# Autodesk Inventor assembly: 305-05
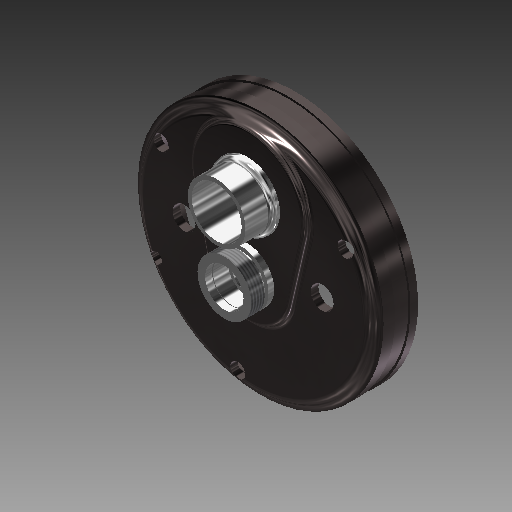
[picture p0: Inventor's stored thumbnail of the model, 512x512]
Saved by Autodesk Inventor 2019 (Build 230136000, 136)
## iProperties
Company: Autodesk Inc.
Created: 2012-01-27
Part Number: 305-05
Document SubType Name: Assembly
Designer: Autodesk Inc.
Mass: 30.5241 g
Surface Area: 116.227 cm^2
Volume: 9.19075 cm^3
Density: 3.32117 g/cm^3
Author: Inventor
## Documents named in this file (4)
- C:\TEMP\Fishing Rod\Workspaces\Handle Side Cover Assembly.iam
- C:\TEMP\Fishing Rod\Workspaces\Handle Side Cover Body.ipt
- C:\TEMP\Fishing Rod\Workspaces\Bearing Housing.ipt
- C:\TEMP\Fishing Rod\Workspaces\Cover Handle Port Sleeve.ipt
## Components (3 placed, 3 different names)
1. Handle Side Cover Body:1 — Insert:1, Insert:2
2. Bearing Housing:1 — Insert:1
3. Cover Handle Port Sleeve:1 — Insert:2
## Relationships (2: Insert 2)
- Insert:1: Handle Side Cover Body:1 ↔ Bearing Housing:1
- Insert:2: Handle Side Cover Body:1 ↔ Cover Handle Port Sleeve:1
